# Autodesk Inventor assembly: A2017_T2_02
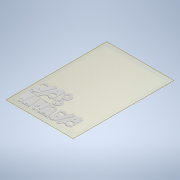
[picture p0: Inventor's stored thumbnail of the model, 180x180]
Saved by Autodesk Inventor 2020 (Build 240168000, 168)
## iProperties
Created: 2021-08-27
Part Number: A2017_T2_02
Document SubType Name: Assembly
Designer: Masato
Author: Masato
## Documents named in this file (6)
- C:\Users\naoki\Documents\Inventor\CitBrains\git_clone\OpenPlatform4_0\CAM\1017_organize\OpenPlatform_ver3_0\cam\A2017_T2_02.iam
- C:\Users\naoki\Documents\Inventor\CitBrains\git_clone\OpenPlatform4_0\CAM\1017_organize\OpenPlatform_ver3_0\cam\Disposable_Board.ipt
- C:\Users\naoki\Documents\Inventor\CitBrains\git_clone\OpenPlatform4_0\CAM\1017_organize\OpenPlatform_ver3_0\UpperBody\Arm\Shoulder_side_frame.ipt
- C:\Users\naoki\Documents\Inventor\CitBrains\git_clone\OpenPlatform4_0\CAM\1017_organize\OpenPlatform_ver3_0\UpperBody\Trunk\Inner_flange.ipt
- C:\Users\naoki\Documents\Inventor\CitBrains\git_clone\OpenPlatform4_0\CAM\1017_organize\OpenPlatform_ver3_0\LowerBody\Foot\Foot_front_frame.ipt
- C:\Users\naoki\Documents\Inventor\CitBrains\git_clone\OpenPlatform4_0\CAM\1017_organize\OpenPlatform_ver3_0\LowerBody\Leg_joit\Leg_joint_pitch_frame.ipt
## Components (11 placed, 5 different names)
1. Disposable_Board:1 — メイト:2, メイト:1, フラッシュ:1, フラッシュ:2, フラッシュ:3, フラッシュ:6, メイト:15, メイト:16, メイト:17
2. Shoulder_side_frame:1 — メイト:4, フラッシュ:3, フラッシュ:4, 正接:1, 正接:2, 正接:3, メイト:12, メイト:13
3. Shoulder_side_frame:2 — メイト:5, 正接:1, メイト:12, 正接:5, 正接:7
4. Foot_front_frame:1 — メイト:6, フラッシュ:4, フラッシュ:5, メイト:11, 正接:5
5. Foot_front_frame:2 — メイト:7, 正接:2, フラッシュ:6, メイト:11, フラッシュ:7, メイト:19
6. Leg_joint_pitch_frame:1 — メイト:8, フラッシュ:5, メイト:13, メイト:14
7. Leg_joint_pitch_frame:2 — メイト:9, 正接:3, メイト:14
8. Leg_joint_pitch_frame:3 — メイト:15, メイト:18, フラッシュ:7, メイト:19, 正接:6
9. Leg_joint_pitch_frame:4 — メイト:16, メイト:18, 正接:6, 正接:8
10. Inner_flange:1 — メイト:17, 正接:7, 正接:8
11. Inner_flange:2
## Component patterns: (2 elements, first: Inner_flange:1)
## Relationships (31: Mate 17, Flush 7, Tangent 7)
- メイト:2 [Mate]: Disposable_Board:1
- メイト:1 [Mate]: Disposable_Board:1
- フラッシュ:1 [Flush]: Disposable_Board:1
- フラッシュ:2 [Flush]: Disposable_Board:1
- メイト:4 [Mate]: Shoulder_side_frame:1
- メイト:5 [Mate]: Shoulder_side_frame:2
- メイト:6 [Mate]: Foot_front_frame:1
- メイト:7 [Mate]: Foot_front_frame:2
- メイト:8 [Mate]: Leg_joint_pitch_frame:1
- メイト:9 [Mate]: Leg_joint_pitch_frame:2
- フラッシュ:3 [Flush] (2 mm): Disposable_Board:1 ↔ Shoulder_side_frame:1
- フラッシュ:4 [Flush]: Shoulder_side_frame:1 ↔ Foot_front_frame:1
- フラッシュ:5 [Flush]: Foot_front_frame:1 ↔ Leg_joint_pitch_frame:1
- 正接:1 [Tangent]: Shoulder_side_frame:1 ↔ Shoulder_side_frame:2
- 正接:2 [Tangent]: Shoulder_side_frame:1 ↔ Foot_front_frame:2
- 正接:3 [Tangent]: Shoulder_side_frame:1 ↔ Leg_joint_pitch_frame:2
- フラッシュ:6 [Flush] (2 mm): Disposable_Board:1 ↔ Foot_front_frame:2
- メイト:11 [Mate] (2.5 mm): Foot_front_frame:1 ↔ Foot_front_frame:2
- メイト:12 [Mate] (2.5 mm): Shoulder_side_frame:1 ↔ Shoulder_side_frame:2
- 正接:5 [Tangent] (3 mm): Shoulder_side_frame:2 ↔ Foot_front_frame:1
- メイト:13 [Mate] (2.5 mm): Shoulder_side_frame:1 ↔ Leg_joint_pitch_frame:1
- メイト:14 [Mate] (2.5 mm): Leg_joint_pitch_frame:1 ↔ Leg_joint_pitch_frame:2
- メイト:15 [Mate]: Disposable_Board:1 ↔ Leg_joint_pitch_frame:3
- メイト:16 [Mate]: Disposable_Board:1 ↔ Leg_joint_pitch_frame:4
- メイト:17 [Mate]: Disposable_Board:1 ↔ Inner_flange:1
- メイト:18 [Mate] (2.5 mm): Leg_joint_pitch_frame:3 ↔ Leg_joint_pitch_frame:4
- フラッシュ:7 [Flush]: Foot_front_frame:2 ↔ Leg_joint_pitch_frame:3
- メイト:19 [Mate] (2.5 mm): Foot_front_frame:2 ↔ Leg_joint_pitch_frame:3
- 正接:6 [Tangent]: Leg_joint_pitch_frame:3 ↔ Leg_joint_pitch_frame:4
- 正接:7 [Tangent] (2.5 mm): Shoulder_side_frame:2 ↔ Inner_flange:1
- 正接:8 [Tangent] (2.5 mm): Leg_joint_pitch_frame:4 ↔ Inner_flange:1
